# Autodesk Inventor assembly: motor_arm
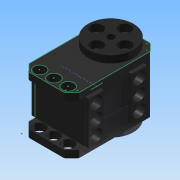
[picture p0: Inventor's stored thumbnail of the model, 180x180]
Saved by Autodesk Inventor 2015 (Build 190159000, 159)
## iProperties
Created: 2016-03-01
Part Number: motor_arm
Document SubType Name: Assembly
Designer: Gregwar
Author: Gregwar
## Documents named in this file (4)
- C:\Users\Gregwar\Desktop\Metabot\3d\autodesk\models\motor_arm.iam
- C:\Users\Gregwar\Desktop\Metabot\3d\autodesk\models\motor.ipt
- C:\Users\Gregwar\Desktop\Metabot\3d\autodesk\models\arm.ipt
- C:\Users\Gregwar\Desktop\Metabot\3d\autodesk\models\counter_arm.ipt
## Components (3 placed, 3 different names)
1. motor:1 — Placage:1, Placage:2, Placage:3, Placage:4
2. arm:1 — Placage:1, Placage:2
3. counter_arm:1 — Placage:3, Placage:4
## Relationships (4: Mate 4)
- Placage:1 [Mate]: motor:1 ↔ arm:1
- Placage:2 [Mate]: motor:1 ↔ arm:1
- Placage:3 [Mate]: motor:1 ↔ counter_arm:1
- Placage:4 [Mate]: motor:1 ↔ counter_arm:1
